# Autodesk Inventor assembly: OpenROV_v2_5_Assembly
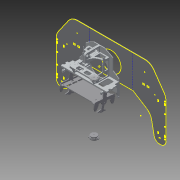
[picture p0: Inventor's stored thumbnail of the model, 180x180]
Saved by Autodesk Inventor 2013 (Build 170138000, 138)
## iProperties
Created: 2013-11-11
Part Number: OpenROV_v2_5_Assembly
Document SubType Name: Assembly
Designer: Eric
Author: Eric
## Documents named in this file (22)
- C:\Users\Eric\Documents\GitHub\openrov-hardware\CAD_Files_OpenROV_v2_5\OpenROV_v2_5_Assembly.iam
- C:\Users\Eric\Documents\GitHub\openrov-hardware\CAD_Files_OpenROV_v2_5\Internal Structure\Bulkhead 25083113.ipt
- C:\Users\Eric\Documents\GitHub\openrov-hardware\CAD_Files_OpenROV_v2_5\Internal Structure\Axial Shroud Support 25090213.ipt
- C:\Users\Eric\Documents\GitHub\openrov-hardware\CAD_Files_OpenROV_v2_5\Internal Structure\Bulkhead Brace 25100613.ipt
- C:\Users\Eric\Documents\GitHub\openrov-hardware\CAD_Files_OpenROV_v2_5\Internal Structure\Vertical Motor Mount 25090213.ipt
- C:\Users\Eric\Documents\GitHub\openrov-hardware\CAD_Files_OpenROV_v2_5\Internal Structure\Horizontal Motor Mount 25090213.ipt
- C:\Users\Eric\Documents\GitHub\openrov-hardware\CAD_Files_OpenROV_v2_5\Internal Structure\Handle 25090213.ipt
- C:\Users\Eric\Documents\GitHub\openrov-hardware\CAD_Files_OpenROV_v2_5\Internal Structure\Lateral Shroud Support 25090213.ipt
- C:\Users\Eric\Documents\GitHub\openrov-hardware\CAD_Files_OpenROV_v2_5\Internal Structure\Top Plate 25090213.ipt
- C:\Users\Eric\Documents\GitHub\openrov-hardware\CAD_Files_OpenROV_v2_5\Internal Structure\Tube Cradle 25090213.ipt
- C:\Users\Eric\Documents\GitHub\openrov-hardware\CAD_Files_OpenROV_v2_5\Battery Pack\Aft Inner Disk.ipt
- C:\Users\Eric\Documents\GitHub\openrov-hardware\CAD_Files_OpenROV_v2_5\Battery Pack\Aft Middle Disk.ipt
- C:\Users\Eric\Documents\GitHub\openrov-hardware\CAD_Files_OpenROV_v2_5\Battery Pack\Aft Outer Disk.ipt
- C:\Users\Eric\Documents\GitHub\openrov-hardware\CAD_Files_OpenROV_v2_5\Battery Pack\Front Large Disk.ipt
- C:\Users\Eric\Documents\GitHub\openrov-hardware\CAD_Files_OpenROV_v2_5\Battery Pack\Front Small Disk.ipt
- C:\Users\Eric\Documents\GitHub\openrov-hardware\CAD_Files_OpenROV_v2_5\Battery Pack\Front Outer Disk.ipt
- C:\Users\Eric\Documents\GitHub\openrov-hardware\CAD_Files_OpenROV_v2_5\E-Chassis\Main_Platform.ipt
- C:\Users\Eric\Documents\GitHub\openrov-hardware\CAD_Files_OpenROV_v2_5\E-Chassis\Endplate.ipt
- C:\Users\Eric\Documents\GitHub\openrov-hardware\CAD_Files_OpenROV_v2_5\E-Chassis\Endplate_Support.ipt
- C:\Users\Eric\Documents\GitHub\openrov-hardware\CAD_Files_OpenROV_v2_5\E-Chassis\Camera_Mount_A.ipt
- C:\Users\Eric\Documents\GitHub\openrov-hardware\CAD_Files_OpenROV_v2_5\E-Chassis\Camera_Mount_B.ipt
- C:\Users\Eric\Documents\GitHub\openrov-hardware\CAD_Files_OpenROV_v2_5\Shell\Shell 25083113.ipt
## Components (34 placed, 21 different names)
1. Bulkhead 25083113:1 — Mate:1, Mate:2, Mate:3, Mate:4, Mate:5, Mate:6, Mate:7, Flush:1, Flush:2, Mate:8, Mate:9, Mate:10, Mate:21, Mate:22, Mate:23, Mate:27, Mate:28, Mate:30, Mate:31
2. Axial Shroud Support 25090213:1 — Mate:1, Mate:2, Mate:3
3. Axial Shroud Support 25090213:2 — Mate:4, Mate:5, Mate:6
4. Bulkhead Brace 25100613:1 — Mate:7, Flush:1, Flush:2
5. Vertical Motor Mount 25090213:1 — Mate:8, Mate:9, Mate:10, Mate:11, Mate:12, Mate:13
6. Horizontal Motor Mount 25090213:1 — Mate:11, Mate:12, Mate:13
7. Handle 25090213:1 — Mate:14, Flush:3, Flush:4, Mate:17
8. Handle 25090213:2 — Mate:14, Flush:3, Flush:4, Mate:15, Flush:5, Flush:6, Mate:16, Mate:18, Mate:19, Flush:7
9. Handle 25090213:3 — Mate:15, Flush:5, Flush:6, Mate:20
10. Lateral Shroud Support 25090213:1 — Mate:16, Mate:17, Mate:18
11. Top Plate 25090213:1 — Mate:19, Flush:7, Mate:20, Mate:21, Mate:22, Mate:23, Mate:26, Mate:29, Flush:14
12. Tube Cradle 25090213:1 — Mate:24, Flush:8, Flush:9
13. Tube Cradle 25090213:2 — Mate:24, Flush:8, Flush:9, Mate:26, Mate:27, Mate:28, Mate:72
14. Tube Cradle 25090213:3 — Mate:25, Flush:10, Flush:11, Mate:29, Mate:30, Mate:31
15. Tube Cradle 25090213:4 — Mate:25, Flush:10, Flush:11
16. Aft Inner Disk:1 — Mate:32, Mate:33, Mate:34, Mate:44, Mate:45
17. Aft Middle Disk:1 — Mate:32, Mate:33, Mate:34, Mate:35, Mate:36, Mate:37
18. Aft Outer Disk:1 — Mate:35, Mate:36, Mate:37
19. Front Large Disk:1 — Mate:40, Mate:41, Mate:42, Mate:43
20. Front Small Disk:1 — Mate:38, Mate:39, Mate:40, Mate:41
21. Front Large Disk:2 — Mate:38, Mate:39, Mate:44, Mate:45
22. Front Outer Disk:1 — Mate:42, Mate:43
23. Main_Platform:1 — Mate:46, Mate:47, Mate:48, Mate:49, Mate:50, Mate:51, Mate:53, Mate:56, Mate:59, Mate:62
24. Endplate:1 — Mate:46, Mate:47, Mate:48, Mate:52, Mate:54, Mate:55, Mate:57, Mate:70, Mate:71
25. Endplate:2 — Mate:49, Mate:50, Mate:51, Mate:58, Mate:60, Mate:61, Mate:63, Mate:68, Mate:69, Mate:72
26. Endplate_Support:1 — Mate:55, Mate:56, Mate:57
27. Endplate_Support:2 — Mate:52, Mate:53, Mate:54
28. Endplate_Support:3 — Mate:61, Mate:62, Mate:63
29. Endplate_Support:4 — Mate:58, Mate:59, Mate:60
30. Camera_Mount_A:1 — Mate:66, Mate:67, Flush:13, Mate:68, Mate:69
31. Camera_Mount_A:2 — Mate:64, Mate:65, Flush:12, Mate:70, Mate:71
32. Camera_Mount_B:1 — Mate:66, Mate:67, Flush:13
33. Camera_Mount_B:2 — Mate:64, Mate:65, Flush:12
34. Shell 25083113:1 — Flush:14
## Relationships (86: Mate 72, Flush 14)
- Mate:1: Bulkhead 25083113:1 ↔ Axial Shroud Support 25090213:1
- Mate:2: Bulkhead 25083113:1 ↔ Axial Shroud Support 25090213:1
- Mate:3: Bulkhead 25083113:1 ↔ Axial Shroud Support 25090213:1
- Mate:4: Bulkhead 25083113:1 ↔ Axial Shroud Support 25090213:2
- Mate:5: Bulkhead 25083113:1 ↔ Axial Shroud Support 25090213:2
- Mate:6: Bulkhead 25083113:1 ↔ Axial Shroud Support 25090213:2
- Mate:7: Bulkhead 25083113:1 ↔ Bulkhead Brace 25100613:1
- Flush:1: Bulkhead 25083113:1 ↔ Bulkhead Brace 25100613:1
- Flush:2: Bulkhead 25083113:1 ↔ Bulkhead Brace 25100613:1
- Mate:8: Bulkhead 25083113:1 ↔ Vertical Motor Mount 25090213:1
- Mate:9: Bulkhead 25083113:1 ↔ Vertical Motor Mount 25090213:1
- Mate:10: Bulkhead 25083113:1 ↔ Vertical Motor Mount 25090213:1
- Mate:11: Vertical Motor Mount 25090213:1 ↔ Horizontal Motor Mount 25090213:1
- Mate:12: Vertical Motor Mount 25090213:1 ↔ Horizontal Motor Mount 25090213:1
- Mate:13: Vertical Motor Mount 25090213:1 ↔ Horizontal Motor Mount 25090213:1
- Mate:14: Handle 25090213:1 ↔ Handle 25090213:2
- Flush:3: Handle 25090213:1 ↔ Handle 25090213:2
- Flush:4: Handle 25090213:1 ↔ Handle 25090213:2
- Mate:15: Handle 25090213:2 ↔ Handle 25090213:3
- Flush:5: Handle 25090213:2 ↔ Handle 25090213:3
- Flush:6: Handle 25090213:2 ↔ Handle 25090213:3
- Mate:16: Handle 25090213:2 ↔ Lateral Shroud Support 25090213:1
- Mate:17: Handle 25090213:1 ↔ Lateral Shroud Support 25090213:1
- Mate:18: Handle 25090213:2 ↔ Lateral Shroud Support 25090213:1
- Mate:19: Handle 25090213:2 ↔ Top Plate 25090213:1
- Flush:7: Handle 25090213:2 ↔ Top Plate 25090213:1
- Mate:20: Handle 25090213:3 ↔ Top Plate 25090213:1
- Mate:21: Bulkhead 25083113:1 ↔ Top Plate 25090213:1
- Mate:22: Bulkhead 25083113:1 ↔ Top Plate 25090213:1
- Mate:23: Bulkhead 25083113:1 ↔ Top Plate 25090213:1
- Mate:24: Tube Cradle 25090213:1 ↔ Tube Cradle 25090213:2
- Flush:8: Tube Cradle 25090213:1 ↔ Tube Cradle 25090213:2
- Flush:9: Tube Cradle 25090213:1 ↔ Tube Cradle 25090213:2
- Mate:25: Tube Cradle 25090213:3 ↔ Tube Cradle 25090213:4
- Flush:10: Tube Cradle 25090213:3 ↔ Tube Cradle 25090213:4
- Flush:11: Tube Cradle 25090213:3 ↔ Tube Cradle 25090213:4
- Mate:26: Top Plate 25090213:1 ↔ Tube Cradle 25090213:2
- Mate:27: Bulkhead 25083113:1 ↔ Tube Cradle 25090213:2
- Mate:28: Bulkhead 25083113:1 ↔ Tube Cradle 25090213:2
- Mate:29: Top Plate 25090213:1 ↔ Tube Cradle 25090213:3
- Mate:30: Bulkhead 25083113:1 ↔ Tube Cradle 25090213:3
- Mate:31: Bulkhead 25083113:1 ↔ Tube Cradle 25090213:3
- Mate:32: Aft Inner Disk:1 ↔ Aft Middle Disk:1
- Mate:33: Aft Inner Disk:1 ↔ Aft Middle Disk:1
- Mate:34: Aft Inner Disk:1 ↔ Aft Middle Disk:1
- Mate:35: Aft Middle Disk:1 ↔ Aft Outer Disk:1
- Mate:36: Aft Middle Disk:1 ↔ Aft Outer Disk:1
- Mate:37: Aft Middle Disk:1 ↔ Aft Outer Disk:1
- Mate:38: Front Small Disk:1 ↔ Front Large Disk:2
- Mate:39: Front Small Disk:1 ↔ Front Large Disk:2
- Mate:40: Front Large Disk:1 ↔ Front Small Disk:1
- Mate:41: Front Large Disk:1 ↔ Front Small Disk:1
- Mate:42: Front Large Disk:1 ↔ Front Outer Disk:1
- Mate:43: Front Large Disk:1 ↔ Front Outer Disk:1
- Mate:44: Aft Inner Disk:1 ↔ Front Large Disk:2
- Mate:45 (218 mm): Aft Inner Disk:1 ↔ Front Large Disk:2
- Mate:46: Main_Platform:1 ↔ Endplate:1
- Mate:47: Main_Platform:1 ↔ Endplate:1
- Mate:48: Main_Platform:1 ↔ Endplate:1
- Mate:49: Main_Platform:1 ↔ Endplate:2
- Mate:50: Main_Platform:1 ↔ Endplate:2
- Mate:51: Main_Platform:1 ↔ Endplate:2
- Mate:52: Endplate:1 ↔ Endplate_Support:2
- Mate:53: Main_Platform:1 ↔ Endplate_Support:2
- Mate:54: Endplate:1 ↔ Endplate_Support:2
- Mate:55: Endplate:1 ↔ Endplate_Support:1
- Mate:56: Main_Platform:1 ↔ Endplate_Support:1
- Mate:57: Endplate:1 ↔ Endplate_Support:1
- Mate:58: Endplate:2 ↔ Endplate_Support:4
- Mate:59: Main_Platform:1 ↔ Endplate_Support:4
- Mate:60: Endplate:2 ↔ Endplate_Support:4
- Mate:61: Endplate:2 ↔ Endplate_Support:3
- Mate:62: Main_Platform:1 ↔ Endplate_Support:3
- Mate:63: Endplate:2 ↔ Endplate_Support:3
- Mate:64: Camera_Mount_A:2 ↔ Camera_Mount_B:2
- Mate:65: Camera_Mount_A:2 ↔ Camera_Mount_B:2
- Flush:12: Camera_Mount_A:2 ↔ Camera_Mount_B:2
- Mate:66: Camera_Mount_A:1 ↔ Camera_Mount_B:1
- Mate:67: Camera_Mount_A:1 ↔ Camera_Mount_B:1
- Flush:13: Camera_Mount_A:1 ↔ Camera_Mount_B:1
- Mate:68: Endplate:2 ↔ Camera_Mount_A:1
- Mate:69: Endplate:2 ↔ Camera_Mount_A:1
- Mate:70: Endplate:1 ↔ Camera_Mount_A:2
- Mate:71: Endplate:1 ↔ Camera_Mount_A:2
- Mate:72: Tube Cradle 25090213:2 ↔ Endplate:2
- Flush:14: Top Plate 25090213:1 ↔ Shell 25083113:1
